# Autodesk Inventor assembly: BRUSH CAGE
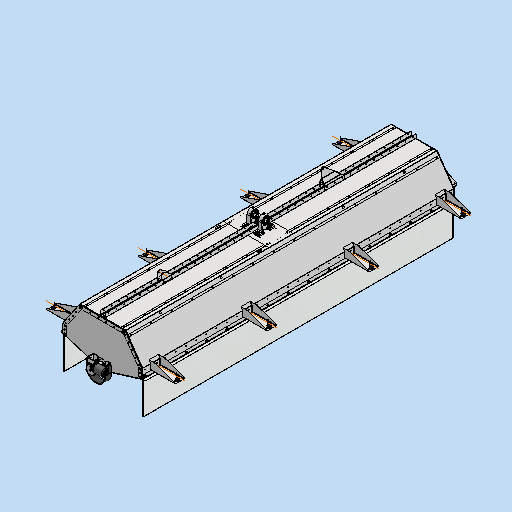
[picture p0: Inventor's stored thumbnail of the model, 512x512]
Saved by Autodesk Inventor 2025.3 (Build 293356030, 356C)
## iProperties
Created: 2025-10-16
Part Number: BRUSH CAGE
Document SubType Name: Assembly
Designer: josh
Mass: 36893.9 g
Surface Area: 125831 cm^2
Volume: 14195.9 cm^3
Density: 2.59891 g/cm^3
Description: BRUSH CAGE COMPLETE, 24" DIAMETER CLEANING BRUSH
Author: josh
## iProperties of the stored document MemberDocs/x12ie5t5mHcoruiwyIxmpz3yaDh
Created: 2025-10-16
Document SubType Name: Assembly
Designer: josh
Mass: 36893.9 g
Surface Area: 125831 cm^2
Volume: 14195.9 cm^3
Density: 2.59891 g/cm^3
Author: josh
## iProperties of the stored document MemberDocs/x01a42iyfB0kmvj1hN3chjb54Ee
Created: 2025-10-16
Document SubType Name: Assembly
Designer: josh
Mass: 36893.9 g
Surface Area: 125831 cm^2
Volume: 14195.9 cm^3
Density: 2.59891 g/cm^3
Author: josh
## iProperties of the stored document MemberDocs/xYuatkekjKkzsr2lw34jfvc5pCb
Created: 2025-10-16
Document SubType Name: Assembly
Designer: josh
Mass: 36893.9 g
Surface Area: 125831 cm^2
Volume: 14195.9 cm^3
Density: 2.59891 g/cm^3
Author: josh
## Documents named in this file (45)
- R:\A1- Neuweg Design Data\OM Robotics\CLEANING BRUSH CAGE & ROLLER\BRUSH CAGE RevC.iam
- R:\A1- Neuweg Design Data\OM Robotics\CLEANING BRUSH CAGE & ROLLER\OM_CAGE-011.ipt
- R:\A1- Neuweg Design Data\OM Robotics\CLEANING BRUSH CAGE & ROLLER\OM_CAGE-012.ipt
- R:\A1- Neuweg Design Data\OM Robotics\CLEANING BRUSH CAGE & ROLLER\OM_CAGE-013.ipt
- R:\A1- Neuweg Design Data\OM Robotics\CLEANING BRUSH CAGE & ROLLER\OM_CAGE-014.ipt
- R:\A1- Neuweg Design Data\OM Robotics\CLEANING BRUSH CAGE & ROLLER\OM_CAGE-015.ipt
- R:\A1- Neuweg Design Data\OM Robotics\CLEANING BRUSH CAGE & ROLLER\OM_CAGE-016.ipt
- R:\A1- Neuweg Design Data\OM Robotics\CLEANING BRUSH CAGE & ROLLER\OM_CAGE-018.ipt
- R:\A1- Neuweg Design Data\OM Robotics\CLEANING BRUSH CAGE & ROLLER\OM_CAGE-019.ipt
- R:\A1- Neuweg Design Data\OM Robotics\CLEANING BRUSH CAGE & ROLLER\OM_CAGE-020.ipt
- R:\A1- Neuweg Design Data\OM Robotics\CLEANING BRUSH CAGE & ROLLER\Shaft Coupler.ipt
- R:\A1- Neuweg Design Data\OM Robotics\CLEANING BRUSH CAGE & ROLLER\SENSOR BRACKET RevC.iam
- R:\A1- Neuweg Design Data\OM Robotics\CLEANING BRUSH CAGE & ROLLER\OM_CAGE-021.ipt
- R:\A1- Neuweg Design Data\OM Robotics\CLEANING BRUSH CAGE & ROLLER\OM_CAGE-022.ipt
- R:\A1- Neuweg Design Data\OM Robotics\CLEANING BRUSH CAGE & ROLLER\OM_CAGE-023.ipt
- R:\A1- Neuweg Design Data\OM Robotics\CLEANING BRUSH CAGE & ROLLER\OM_CAGE-024.ipt
- R:\A1- Neuweg Design Data\OM Robotics\CLEANING BRUSH CAGE & ROLLER\4453N16.ipt
- R:\A1- Neuweg Design Data\OM Robotics\CLEANING BRUSH CAGE & ROLLER\UCFL205-16_Simplify.ipt
- R:\A1- Neuweg Design Data\OM Robotics\CLEANING BRUSH CAGE & ROLLER\BRUSH TUBE_RevA.iam
- R:\A1- Neuweg Design Data\OM Robotics\CLEANING BRUSH CAGE & ROLLER\218-2002_Simplify.ipt
- R:\A1- Neuweg Design Data\OM Robotics\CLEANING BRUSH CAGE & ROLLER\94842A101.ipt
- R:\A1- Neuweg Design Data\OM Robotics\CLEANING BRUSH CAGE & ROLLER\95031A124.ipt
- R:\A1- Neuweg Design Data\OM Robotics\CLEANING BRUSH CAGE & ROLLER\Fan Bracket.ipt
- R:\A1- Neuweg Design Data\OM Robotics\CLEANING BRUSH CAGE & ROLLER\98778A541.ipt
- C:\WORK\INVENTOR PROJECTS\misc custom projects\O&M ROBOTICS\OM_CAGE-011.ipt
- C:\WORK\INVENTOR PROJECTS\misc custom projects\O&M ROBOTICS\OM_CAGE-012.ipt
- C:\WORK\INVENTOR PROJECTS\misc custom projects\O&M ROBOTICS\OM_CAGE-013.ipt
- C:\WORK\INVENTOR PROJECTS\misc custom projects\O&M ROBOTICS\OM_CAGE-014.ipt
- C:\WORK\INVENTOR PROJECTS\misc custom projects\O&M ROBOTICS\OM_CAGE-015.ipt
- C:\WORK\INVENTOR PROJECTS\misc custom projects\O&M ROBOTICS\OM_CAGE-016.ipt
- C:\WORK\INVENTOR PROJECTS\misc custom projects\O&M ROBOTICS\OM_CAGE-018.ipt
- C:\WORK\INVENTOR PROJECTS\misc custom projects\O&M ROBOTICS\OM_CAGE-019.ipt
- C:\WORK\INVENTOR PROJECTS\misc custom projects\O&M ROBOTICS\OM_CAGE-020.ipt
- C:\WORK\INVENTOR PROJECTS\misc custom projects\O&M ROBOTICS\ucfl205-16\ucfl205-16\ucfl205-16.iam
- C:\WORK\INVENTOR PROJECTS\misc custom projects\O&M ROBOTICS\BRUSH TUBE_RevA.iam
- C:\WORK\INVENTOR PROJECTS\misc custom projects\O&M ROBOTICS\Shaft Coupler.ipt
- C:\WORK\INVENTOR PROJECTS\misc custom projects\O&M ROBOTICS\218-2002\218-2002\218-2002.iam
- C:\WORK\INVENTOR PROJECTS\misc custom projects\O&M ROBOTICS\SENSOR BRACKET RevC.iam
- C:\WORK\INVENTOR PROJECTS\misc custom projects\O&M ROBOTICS\ucpa205-16\ucpa205-16\ucpa205-16.iam
- C:\WORK\INVENTOR PROJECTS\misc custom projects\O&M ROBOTICS\OM_CAGE-021.ipt
- C:\WORK\INVENTOR PROJECTS\misc custom projects\O&M ROBOTICS\Fan+Bracket.iam
- C:\WORK\INVENTOR PROJECTS\misc custom projects\O&M ROBOTICS\4453N16_Extra-Clearance Mounted Ball Bearing.ipt
- C:\WORK\INVENTOR PROJECTS\misc custom projects\O&M ROBOTICS\OM_CAGE-022.ipt
- C:\WORK\INVENTOR PROJECTS\misc custom projects\O&M ROBOTICS\OM_CAGE-023.ipt
- C:\WORK\INVENTOR PROJECTS\misc custom projects\O&M ROBOTICS\OM_CAGE-024.ipt
## Components (228 placed, 23 different names)
1. OM_CAGE-011:1 — Mate:4, Mate:5, Mate:6, Mate:8, Mate:10, Mate:11, Mate:18, Mate:17, Insert:16, Insert:17, Mate:20, Mate:22, Mate:23, Mate:24, Mate:25, Mate:26, Mate:27, Mate:28, Mate:29, Mate:30, Mate:31, Mate:32, Mate:33, Mate:34, Mate:35, Insert:95, Insert:96, Insert:97, Insert:98, Insert:99, Insert:100, Insert:101, Insert:102, Insert:103, Insert:104, Insert:105, Insert:106, Insert:107, Insert:108, Insert:109, Insert:110, Insert:111, Insert:112, Insert:113, Insert:114, Insert:115, Insert:116, Insert:117, Insert:118, Insert:119, Insert:120, Insert:121, Insert:122, Insert:123, Insert:124, Insert:125, Insert:126, Insert:127, Insert:128, Insert:129, Insert:130, Insert:131, Insert:132, Insert:133, Insert:134, Insert:135, Insert:136, Insert:137, Insert:138, Insert:139, Insert:140, Insert:141, Insert:142, Insert:143, Insert:144, Insert:145, Insert:146, Insert:147, Insert:148, Insert:149, Insert:150, Insert:151, Insert:152, Insert:153, Insert:154, Insert:155, Insert:156, Insert:157, Insert:158, Insert:159, Insert:160, Insert:161, Insert:162, Insert:163, Insert:164, Insert:165, Insert:166, Insert:167, Insert:168, Insert:169, Insert:170, Insert:171, Insert:172, Insert:173, Insert:174, Insert:175, Insert:176, Insert:177, Insert:178, Insert:179, Insert:180, Insert:181, Insert:182, Insert:183, Insert:184, Insert:185, Insert:186, Insert:187, Insert:188, Insert:189, Insert:190
2. OM_CAGE-012:1 — Insert:25, Insert:26, Insert:31, Insert:32, Insert:33, Insert:34, Insert:35, Insert:36, Insert:37, Insert:38, Insert:39, Insert:40, Insert:41, Insert:42, Insert:43, Insert:44, Insert:45, Insert:46, Insert:47, Insert:48, Insert:49, Insert:50, Insert:51, Insert:52
3. OM_CAGE-013:1 — Mate:15, Insert:12, Insert:13, Mate:16, Mate:19, Insert:20, Insert:21, Insert:23, Insert:24, Insert:75, Insert:76, Insert:77, Insert:78, Insert:79, Insert:80, Insert:81, Insert:82, Insert:83, Insert:84, Insert:85, Insert:86, Insert:87, Insert:88, Insert:89, Insert:90, Insert:91, Insert:92, Insert:93, Insert:94
4. OM_CAGE-014:1
5. OM_CAGE-015:1
6. OM_CAGE-016:1 — Insert:191, Insert:192, Insert:193, Insert:194, Insert:195, Insert:196, Insert:197, Insert:198, Insert:199, Insert:200, Insert:201, Insert:202, Insert:203, Insert:204, Insert:205, Insert:206
7. OM_CAGE-018:1 — Insert:11
8. OM_CAGE-019:1 — Mate:36, Insert:27, Insert:28, Insert:53, Insert:54, Insert:55, Insert:56, Insert:57, Insert:58, Insert:59, Insert:60, Insert:61, Insert:62, Insert:63, Insert:64, Insert:65, Insert:66, Insert:67, Insert:68, Insert:69, Insert:70, Insert:71, Insert:72, Insert:73, Insert:74, Flush:2, Mate:39, Mate:40, Mate:41, Mate:42, Mate:43
9. OM_CAGE-020:1
10. OM_CAGE-018:2
11. OM_CAGE-020:2
12. OM_CAGE-015:2
13. OM_CAGE-016:2 — Insert:207, Insert:208, Insert:209, Insert:210, Insert:211, Insert:212, Insert:213, Insert:214, Insert:215, Insert:216, Insert:217, Insert:218, Insert:219, Insert:220, Insert:221, Insert:222
14. UCFL205-16_Simplify:1 — Insert:25, Insert:26, Insert:29
15. UCFL205-16_Simplify:2 — Mate:36, Insert:27, Insert:28, Mate:37
16. Shaft Coupler:1 — Mate:3, Mate:38, Insert:30
17. 218-2002_Simplify:1 — Mate:3, Insert:11
18. SENSOR BRACKET RevC:1 [sub-assembly] — Mate:4, Mate:5
19. SENSOR BRACKET RevC:2 [sub-assembly] — Mate:6, Mate:26, Mate:27
20. SENSOR BRACKET RevC:3 [sub-assembly] — Mate:10, Mate:11, Mate:24, Mate:25
21. SENSOR BRACKET RevC:4 [sub-assembly] — Mate:8, Mate:22, Mate:23
22. SENSOR BRACKET RevC:5 [sub-assembly] — Mate:31, Mate:32
23. SENSOR BRACKET RevC:6 [sub-assembly] — Mate:30, Mate:33
24. SENSOR BRACKET RevC:7 [sub-assembly] — Mate:28, Mate:35
25. SENSOR BRACKET RevC:8 [sub-assembly] — Mate:29, Mate:34
26. OM_CAGE-021:1 — Mate:14, Flush:1, Insert:12, Insert:13
27. OM_CAGE-021:2 — Mate:14, Mate:15, Flush:1
28. Fan Bracket:1 — Flush:2, Mate:40, Mate:43
29. Fan Bracket:2 — Mate:39, Mate:41, Mate:42
30. 4453N16:1 — Mate:16, Mate:18, Mate:17, Mate:19, Mate:21
31. OM_CAGE-022:1
32. OM_CAGE-022:2 — Insert:16, Insert:17
33. 4453N16:2 — Mate:20, Mate:21
34. OM_CAGE-023:1 — Insert:20, Insert:21, Insert:22
35. OM_CAGE-024:1 — Insert:22, Insert:23, Insert:24
36. BRUSH TUBE_RevA:1 [sub-assembly] — Insert:29, Mate:37, Mate:38, Insert:30
37. 98778A541:1 — Insert:31
38. 98778A541:2 — Insert:32
39. 98778A541:3 — Insert:33
40. 98778A541:4 — Insert:34
41. 98778A541:5 — Insert:35
42. 98778A541:6 — Insert:36
43. 98778A541:7 — Insert:37
44. 98778A541:8 — Insert:38
45. 98778A541:9 — Insert:39
46. 98778A541:10 — Insert:40
47. 98778A541:11 — Insert:41
48. 98778A541:12 — Insert:42
49. 98778A541:13 — Insert:43
50. 98778A541:14 — Insert:44
51. 98778A541:15 — Insert:45
52. 98778A541:16 — Insert:46
53. 98778A541:17 — Insert:47
54. 98778A541:18 — Insert:48
55. 98778A541:19 — Insert:49
56. 98778A541:20 — Insert:50
57. 98778A541:21 — Insert:51
58. 98778A541:22 — Insert:52
59. 98778A541:23 — Insert:53
60. 98778A541:24 — Insert:54
61. 98778A541:25 — Insert:55
62. 98778A541:26 — Insert:56
63. 98778A541:27 — Insert:57
64. 98778A541:28 — Insert:58
65. 98778A541:29 — Insert:59
66. 98778A541:30 — Insert:60
67. 98778A541:31 — Insert:61
68. 98778A541:32 — Insert:62
69. 98778A541:33 — Insert:63
70. 98778A541:34 — Insert:64
71. 98778A541:35 — Insert:65
72. 98778A541:36 — Insert:66
73. 98778A541:37 — Insert:67
74. 98778A541:38 — Insert:68
75. 98778A541:39 — Insert:69
76. 98778A541:40 — Insert:70
77. 98778A541:41 — Insert:71
78. 98778A541:42 — Insert:72
79. 98778A541:43 — Insert:73
80. 98778A541:44 — Insert:74
81. 98778A541:45 — Insert:75
82. 98778A541:46 — Insert:76
83. 98778A541:47 — Insert:77
84. 98778A541:48 — Insert:78
85. 98778A541:49 — Insert:79
86. 98778A541:50 — Insert:80
87. 98778A541:51 — Insert:81
88. 98778A541:52 — Insert:82
89. 98778A541:53 — Insert:83
90. 98778A541:54 — Insert:84
91. 98778A541:55 — Insert:85
92. 98778A541:56 — Insert:86
93. 98778A541:57 — Insert:87
94. 98778A541:58 — Insert:88
95. 98778A541:59 — Insert:89
96. 98778A541:60 — Insert:90
97. 98778A541:61 — Insert:91
98. 98778A541:62 — Insert:92
99. 98778A541:63 — Insert:93
100. 98778A541:64 — Insert:94
101. 98778A541:65 — Insert:95
102. 98778A541:66 — Insert:96
103. 98778A541:67 — Insert:97
104. 98778A541:68 — Insert:98
105. 98778A541:69 — Insert:99
106. 98778A541:70 — Insert:100
107. 98778A541:71 — Insert:101
108. 98778A541:72 — Insert:102
109. 98778A541:73 — Insert:103
110. 98778A541:74 — Insert:104
111. 98778A541:75 — Insert:105
112. 98778A541:76 — Insert:106
113. 98778A541:77 — Insert:107
114. 98778A541:78 — Insert:108
115. 98778A541:79 — Insert:109
116. 98778A541:80 — Insert:110
117. 98778A541:81 — Insert:111
118. 98778A541:82 — Insert:112
119. 98778A541:83 — Insert:113
120. 98778A541:84 — Insert:114
121. 98778A541:85 — Insert:115
122. 98778A541:86 — Insert:116
123. 98778A541:87 — Insert:117
124. 98778A541:88 — Insert:118
125. 98778A541:89 — Insert:119
126. 98778A541:90 — Insert:120
127. 98778A541:91 — Insert:121
128. 98778A541:92 — Insert:122
129. 98778A541:93 — Insert:123
130. 98778A541:94 — Insert:124
131. 98778A541:95 — Insert:125
132. 98778A541:96 — Insert:126
133. 98778A541:97 — Insert:127
134. 98778A541:98 — Insert:128
135. 98778A541:99 — Insert:129
136. 98778A541:100 — Insert:130
137. 98778A541:101 — Insert:131
138. 98778A541:102 — Insert:132
139. 98778A541:103 — Insert:133
140. 98778A541:104 — Insert:134
141. 98778A541:105 — Insert:135
142. 98778A541:106 — Insert:136
143. 98778A541:107 — Insert:137
144. 98778A541:108 — Insert:138
145. 98778A541:109 — Insert:139
146. 98778A541:110 — Insert:140
147. 98778A541:111 — Insert:141
148. 98778A541:112 — Insert:142
149. 98778A541:113 — Insert:143
150. 98778A541:114 — Insert:144
151. 98778A541:115 — Insert:145
152. 98778A541:116 — Insert:146
153. 98778A541:117 — Insert:147
154. 98778A541:118 — Insert:148
155. 98778A541:119 — Insert:149
156. 98778A541:120 — Insert:150
157. 98778A541:121 — Insert:151
158. 98778A541:122 — Insert:152
159. 98778A541:123 — Insert:153
160. 98778A541:124 — Insert:154
161. 98778A541:125 — Insert:155
162. 98778A541:126 — Insert:156
163. 98778A541:127 — Insert:157
164. 98778A541:128 — Insert:158
165. 94842A101:1 — Insert:159
166. 94842A101:2 — Insert:160
167. 94842A101:3 — Insert:161
168. 94842A101:4 — Insert:162
169. 94842A101:5 — Insert:163
170. 94842A101:6 — Insert:164
171. 94842A101:7 — Insert:165
172. 94842A101:8 — Insert:166
173. 94842A101:9 — Insert:167
174. 94842A101:10 — Insert:168
175. 94842A101:11 — Insert:169
176. 94842A101:12 — Insert:170
177. 94842A101:13 — Insert:171
178. 94842A101:14 — Insert:172
179. 94842A101:15 — Insert:173
180. 94842A101:16 — Insert:174
181. 94842A101:17 — Insert:175
182. 94842A101:18 — Insert:176
183. 94842A101:19 — Insert:177
184. 94842A101:20 — Insert:178
185. 94842A101:21 — Insert:179
186. 94842A101:22 — Insert:180
187. 94842A101:23 — Insert:181
188. 94842A101:24 — Insert:182
189. 94842A101:25 — Insert:183
190. 94842A101:26 — Insert:184
191. 94842A101:27 — Insert:185
192. 94842A101:28 — Insert:186
193. 94842A101:29 — Insert:187
194. 94842A101:30 — Insert:188
195. 94842A101:31 — Insert:189
196. 94842A101:32 — Insert:190
197. 95031A124:1 — Insert:191
198. 95031A124:2 — Insert:192
199. 95031A124:3 — Insert:193
200. 95031A124:4 — Insert:194
201. 95031A124:5 — Insert:195
202. 95031A124:6 — Insert:196
203. 95031A124:7 — Insert:197
204. 95031A124:8 — Insert:198
205. 95031A124:9 — Insert:199
206. 95031A124:10 — Insert:200
207. 95031A124:11 — Insert:201
208. 95031A124:12 — Insert:202
209. 95031A124:13 — Insert:203
210. 95031A124:14 — Insert:204
211. 95031A124:15 — Insert:205
212. 95031A124:16 — Insert:206
213. 95031A124:17 — Insert:207
214. 95031A124:18 — Insert:208
215. 95031A124:19 — Insert:209
216. 95031A124:20 — Insert:210
217. 95031A124:21 — Insert:211
218. 95031A124:22 — Insert:212
219. 95031A124:23 — Insert:213
220. 95031A124:24 — Insert:214
221. 95031A124:25 — Insert:215
222. 95031A124:26 — Insert:216
223. 95031A124:27 — Insert:217
224. 95031A124:28 — Insert:218
225. 95031A124:29 — Insert:219
226. 95031A124:30 — Insert:220
227. 95031A124:31 — Insert:221
228. 95031A124:32 — Insert:222
## Relationships (247: Insert 208, Mate 37, Flush 2)
- Mate:3: Shaft Coupler:1 ↔ 218-2002_Simplify:1
- Mate:4: OM_CAGE-011:1 ↔ SENSOR BRACKET RevC:1
- Mate:5: OM_CAGE-011:1 ↔ SENSOR BRACKET RevC:1
- Mate:6: OM_CAGE-011:1 ↔ SENSOR BRACKET RevC:2
- Mate:8: OM_CAGE-011:1 ↔ SENSOR BRACKET RevC:4
- Mate:10: OM_CAGE-011:1 ↔ SENSOR BRACKET RevC:3
- Mate:11: OM_CAGE-011:1 ↔ SENSOR BRACKET RevC:3
- Insert:11: OM_CAGE-018:1 ↔ 218-2002_Simplify:1
- Mate:14: OM_CAGE-021:1 ↔ OM_CAGE-021:2
- Mate:15: OM_CAGE-013:1 ↔ OM_CAGE-021:2
- Flush:1: OM_CAGE-021:1 ↔ OM_CAGE-021:2
- Insert:12: OM_CAGE-013:1 ↔ OM_CAGE-021:1
- Insert:13: OM_CAGE-013:1 ↔ OM_CAGE-021:1
- Mate:16: OM_CAGE-013:1 ↔ 4453N16:1
- Mate:18: OM_CAGE-011:1 ↔ 4453N16:1
- Mate:17: OM_CAGE-011:1 ↔ 4453N16:1
- Mate:19 (0.3556 mm): OM_CAGE-013:1 ↔ 4453N16:1
- Insert:16: OM_CAGE-011:1 ↔ OM_CAGE-022:2
- Insert:17: OM_CAGE-011:1 ↔ OM_CAGE-022:2
- Mate:20: OM_CAGE-011:1 ↔ 4453N16:2
- Mate:21: 4453N16:1 ↔ 4453N16:2
- Mate:22: OM_CAGE-011:1 ↔ SENSOR BRACKET RevC:4
- Mate:23: OM_CAGE-011:1 ↔ SENSOR BRACKET RevC:4
- Mate:24: OM_CAGE-011:1 ↔ SENSOR BRACKET RevC:3
- Mate:25: OM_CAGE-011:1 ↔ SENSOR BRACKET RevC:3
- Mate:26: OM_CAGE-011:1 ↔ SENSOR BRACKET RevC:2
- Mate:27: OM_CAGE-011:1 ↔ SENSOR BRACKET RevC:2
- Mate:28: OM_CAGE-011:1 ↔ SENSOR BRACKET RevC:7
- Mate:29: OM_CAGE-011:1 ↔ SENSOR BRACKET RevC:8
- Mate:30: OM_CAGE-011:1 ↔ SENSOR BRACKET RevC:6
- Mate:31: OM_CAGE-011:1 ↔ SENSOR BRACKET RevC:5
- Mate:32: OM_CAGE-011:1 ↔ SENSOR BRACKET RevC:5
- Mate:33: OM_CAGE-011:1 ↔ SENSOR BRACKET RevC:6
- Mate:34: OM_CAGE-011:1 ↔ SENSOR BRACKET RevC:8
- Mate:35: OM_CAGE-011:1 ↔ SENSOR BRACKET RevC:7
- Insert:20: OM_CAGE-013:1 ↔ OM_CAGE-023:1
- Insert:21: OM_CAGE-013:1 ↔ OM_CAGE-023:1
- Insert:22: OM_CAGE-023:1 ↔ OM_CAGE-024:1
- Insert:23: OM_CAGE-013:1 ↔ OM_CAGE-024:1
- Insert:24: OM_CAGE-013:1 ↔ OM_CAGE-024:1
- Insert:25: OM_CAGE-012:1 ↔ UCFL205-16_Simplify:1
- Mate:36: OM_CAGE-019:1 ↔ UCFL205-16_Simplify:2
- Insert:26: OM_CAGE-012:1 ↔ UCFL205-16_Simplify:1
- Insert:27: OM_CAGE-019:1 ↔ UCFL205-16_Simplify:2
- Insert:28: OM_CAGE-019:1 ↔ UCFL205-16_Simplify:2
- Insert:29 (1.5875 mm): UCFL205-16_Simplify:1 ↔ BRUSH TUBE_RevA:1
- Mate:37: UCFL205-16_Simplify:2 ↔ BRUSH TUBE_RevA:1
- Mate:38: Shaft Coupler:1 ↔ BRUSH TUBE_RevA:1
- Insert:30: Shaft Coupler:1 ↔ BRUSH TUBE_RevA:1
- Insert:31: OM_CAGE-012:1 ↔ 98778A541:1
- Insert:32: OM_CAGE-012:1 ↔ 98778A541:2
- Insert:33: OM_CAGE-012:1 ↔ 98778A541:3
- Insert:34: OM_CAGE-012:1 ↔ 98778A541:4
- Insert:35: OM_CAGE-012:1 ↔ 98778A541:5
- Insert:36: OM_CAGE-012:1 ↔ 98778A541:6
- Insert:37: OM_CAGE-012:1 ↔ 98778A541:7
- Insert:38: OM_CAGE-012:1 ↔ 98778A541:8
- Insert:39: OM_CAGE-012:1 ↔ 98778A541:9
- Insert:40: OM_CAGE-012:1 ↔ 98778A541:10
- Insert:41: OM_CAGE-012:1 ↔ 98778A541:11
- Insert:42: OM_CAGE-012:1 ↔ 98778A541:12
- Insert:43: OM_CAGE-012:1 ↔ 98778A541:13
- Insert:44: OM_CAGE-012:1 ↔ 98778A541:14
- Insert:45: OM_CAGE-012:1 ↔ 98778A541:15
- Insert:46: OM_CAGE-012:1 ↔ 98778A541:16
- Insert:47: OM_CAGE-012:1 ↔ 98778A541:17
- Insert:48: OM_CAGE-012:1 ↔ 98778A541:18
- Insert:49: OM_CAGE-012:1 ↔ 98778A541:19
- Insert:50: OM_CAGE-012:1 ↔ 98778A541:20
- Insert:51: OM_CAGE-012:1 ↔ 98778A541:21
- Insert:52: OM_CAGE-012:1 ↔ 98778A541:22
- Insert:53: OM_CAGE-019:1 ↔ 98778A541:23
- Insert:54: OM_CAGE-019:1 ↔ 98778A541:24
- Insert:55: OM_CAGE-019:1 ↔ 98778A541:25
- Insert:56: OM_CAGE-019:1 ↔ 98778A541:26
- Insert:57: OM_CAGE-019:1 ↔ 98778A541:27
- Insert:58: OM_CAGE-019:1 ↔ 98778A541:28
- Insert:59: OM_CAGE-019:1 ↔ 98778A541:29
- Insert:60: OM_CAGE-019:1 ↔ 98778A541:30
- Insert:61: OM_CAGE-019:1 ↔ 98778A541:31
- Insert:62: OM_CAGE-019:1 ↔ 98778A541:32
- Insert:63: OM_CAGE-019:1 ↔ 98778A541:33
- Insert:64: OM_CAGE-019:1 ↔ 98778A541:34
- Insert:65: OM_CAGE-019:1 ↔ 98778A541:35
- Insert:66: OM_CAGE-019:1 ↔ 98778A541:36
- Insert:67: OM_CAGE-019:1 ↔ 98778A541:37
- Insert:68: OM_CAGE-019:1 ↔ 98778A541:38
- Insert:69: OM_CAGE-019:1 ↔ 98778A541:39
- Insert:70: OM_CAGE-019:1 ↔ 98778A541:40
- Insert:71: OM_CAGE-019:1 ↔ 98778A541:41
- Insert:72: OM_CAGE-019:1 ↔ 98778A541:42
- Insert:73: OM_CAGE-019:1 ↔ 98778A541:43
- Insert:74: OM_CAGE-019:1 ↔ 98778A541:44
- Insert:75: OM_CAGE-013:1 ↔ 98778A541:45
- Insert:76: OM_CAGE-013:1 ↔ 98778A541:46
- Insert:77: OM_CAGE-013:1 ↔ 98778A541:47
- Insert:78: OM_CAGE-013:1 ↔ 98778A541:48
- Insert:79: OM_CAGE-013:1 ↔ 98778A541:49
- Insert:80: OM_CAGE-013:1 ↔ 98778A541:50
- Insert:81: OM_CAGE-013:1 ↔ 98778A541:51
- Insert:82: OM_CAGE-013:1 ↔ 98778A541:52
- Insert:83: OM_CAGE-013:1 ↔ 98778A541:53
- Insert:84: OM_CAGE-013:1 ↔ 98778A541:54
- Insert:85: OM_CAGE-013:1 ↔ 98778A541:55
- Insert:86: OM_CAGE-013:1 ↔ 98778A541:56
- Insert:87: OM_CAGE-013:1 ↔ 98778A541:57
- Insert:88: OM_CAGE-013:1 ↔ 98778A541:58
- Insert:89: OM_CAGE-013:1 ↔ 98778A541:59
- Insert:90: OM_CAGE-013:1 ↔ 98778A541:60
- Insert:91: OM_CAGE-013:1 ↔ 98778A541:61
- Insert:92: OM_CAGE-013:1 ↔ 98778A541:62
- Insert:93: OM_CAGE-013:1 ↔ 98778A541:63
- Insert:94: OM_CAGE-013:1 ↔ 98778A541:64
- Insert:95: OM_CAGE-011:1 ↔ 98778A541:65
- Insert:96: OM_CAGE-011:1 ↔ 98778A541:66
- Insert:97: OM_CAGE-011:1 ↔ 98778A541:67
- Insert:98: OM_CAGE-011:1 ↔ 98778A541:68
- Insert:99: OM_CAGE-011:1 ↔ 98778A541:69
- Insert:100: OM_CAGE-011:1 ↔ 98778A541:70
- Insert:101: OM_CAGE-011:1 ↔ 98778A541:71
- Insert:102: OM_CAGE-011:1 ↔ 98778A541:72
- Insert:103: OM_CAGE-011:1 ↔ 98778A541:73
- Insert:104: OM_CAGE-011:1 ↔ 98778A541:74
- Insert:105: OM_CAGE-011:1 ↔ 98778A541:75
- Insert:106: OM_CAGE-011:1 ↔ 98778A541:76
- Insert:107: OM_CAGE-011:1 ↔ 98778A541:77
- Insert:108: OM_CAGE-011:1 ↔ 98778A541:78
- Insert:109: OM_CAGE-011:1 ↔ 98778A541:79
- Insert:110: OM_CAGE-011:1 ↔ 98778A541:80
- Insert:111: OM_CAGE-011:1 ↔ 98778A541:81
- Insert:112: OM_CAGE-011:1 ↔ 98778A541:82
- Insert:113: OM_CAGE-011:1 ↔ 98778A541:83
- Insert:114: OM_CAGE-011:1 ↔ 98778A541:84
- Insert:115: OM_CAGE-011:1 ↔ 98778A541:85
- Insert:116: OM_CAGE-011:1 ↔ 98778A541:86
- Insert:117: OM_CAGE-011:1 ↔ 98778A541:87
- Insert:118: OM_CAGE-011:1 ↔ 98778A541:88
- Insert:119: OM_CAGE-011:1 ↔ 98778A541:89
- Insert:120: OM_CAGE-011:1 ↔ 98778A541:90
- Insert:121: OM_CAGE-011:1 ↔ 98778A541:91
- Insert:122: OM_CAGE-011:1 ↔ 98778A541:92
- Insert:123: OM_CAGE-011:1 ↔ 98778A541:93
- Insert:124: OM_CAGE-011:1 ↔ 98778A541:94
- Insert:125: OM_CAGE-011:1 ↔ 98778A541:95
- Insert:126: OM_CAGE-011:1 ↔ 98778A541:96
- Insert:127: OM_CAGE-011:1 ↔ 98778A541:97
- Insert:128: OM_CAGE-011:1 ↔ 98778A541:98
- Insert:129: OM_CAGE-011:1 ↔ 98778A541:99
- Insert:130: OM_CAGE-011:1 ↔ 98778A541:100
- Insert:131: OM_CAGE-011:1 ↔ 98778A541:101
- Insert:132: OM_CAGE-011:1 ↔ 98778A541:102
- Insert:133: OM_CAGE-011:1 ↔ 98778A541:103
- Insert:134: OM_CAGE-011:1 ↔ 98778A541:104
- Insert:135: OM_CAGE-011:1 ↔ 98778A541:105
- Insert:136: OM_CAGE-011:1 ↔ 98778A541:106
- Insert:137: OM_CAGE-011:1 ↔ 98778A541:107
- Insert:138: OM_CAGE-011:1 ↔ 98778A541:108
- Insert:139: OM_CAGE-011:1 ↔ 98778A541:109
- Insert:140: OM_CAGE-011:1 ↔ 98778A541:110
- Insert:141: OM_CAGE-011:1 ↔ 98778A541:111
- Insert:142: OM_CAGE-011:1 ↔ 98778A541:112
- Insert:143: OM_CAGE-011:1 ↔ 98778A541:113
- Insert:144: OM_CAGE-011:1 ↔ 98778A541:114
- Insert:145: OM_CAGE-011:1 ↔ 98778A541:115
- Insert:146: OM_CAGE-011:1 ↔ 98778A541:116
- Insert:147: OM_CAGE-011:1 ↔ 98778A541:117
- Insert:148: OM_CAGE-011:1 ↔ 98778A541:118
- Insert:149: OM_CAGE-011:1 ↔ 98778A541:119
- Insert:150: OM_CAGE-011:1 ↔ 98778A541:120
- Insert:151: OM_CAGE-011:1 ↔ 98778A541:121
- Insert:152: OM_CAGE-011:1 ↔ 98778A541:122
- Insert:153: OM_CAGE-011:1 ↔ 98778A541:123
- Insert:154: OM_CAGE-011:1 ↔ 98778A541:124
- Insert:155: OM_CAGE-011:1 ↔ 98778A541:125
- Insert:156: OM_CAGE-011:1 ↔ 98778A541:126
- Insert:157: OM_CAGE-011:1 ↔ 98778A541:127
- Insert:158: OM_CAGE-011:1 ↔ 98778A541:128
- Insert:159: OM_CAGE-011:1 ↔ 94842A101:1
- Insert:160: OM_CAGE-011:1 ↔ 94842A101:2
- Insert:161: OM_CAGE-011:1 ↔ 94842A101:3
- Insert:162: OM_CAGE-011:1 ↔ 94842A101:4
- Insert:163: OM_CAGE-011:1 ↔ 94842A101:5
- Insert:164: OM_CAGE-011:1 ↔ 94842A101:6
- Insert:165: OM_CAGE-011:1 ↔ 94842A101:7
- Insert:166: OM_CAGE-011:1 ↔ 94842A101:8
- Insert:167: OM_CAGE-011:1 ↔ 94842A101:9
- Insert:168: OM_CAGE-011:1 ↔ 94842A101:10
- Insert:169: OM_CAGE-011:1 ↔ 94842A101:11
- Insert:170: OM_CAGE-011:1 ↔ 94842A101:12
- Insert:171: OM_CAGE-011:1 ↔ 94842A101:13
- Insert:172: OM_CAGE-011:1 ↔ 94842A101:14
- Insert:173: OM_CAGE-011:1 ↔ 94842A101:15
- Insert:174: OM_CAGE-011:1 ↔ 94842A101:16
- Insert:175: OM_CAGE-011:1 ↔ 94842A101:17
- Insert:176: OM_CAGE-011:1 ↔ 94842A101:18
- Insert:177: OM_CAGE-011:1 ↔ 94842A101:19
- Insert:178: OM_CAGE-011:1 ↔ 94842A101:20
- Insert:179: OM_CAGE-011:1 ↔ 94842A101:21
- Insert:180: OM_CAGE-011:1 ↔ 94842A101:22
- Insert:181: OM_CAGE-011:1 ↔ 94842A101:23
- Insert:182: OM_CAGE-011:1 ↔ 94842A101:24
- Insert:183: OM_CAGE-011:1 ↔ 94842A101:25
- Insert:184: OM_CAGE-011:1 ↔ 94842A101:26
- Insert:185: OM_CAGE-011:1 ↔ 94842A101:27
- Insert:186: OM_CAGE-011:1 ↔ 94842A101:28
- Insert:187: OM_CAGE-011:1 ↔ 94842A101:29
- Insert:188: OM_CAGE-011:1 ↔ 94842A101:30
- Insert:189: OM_CAGE-011:1 ↔ 94842A101:31
- Insert:190: OM_CAGE-011:1 ↔ 94842A101:32
- Insert:191: OM_CAGE-016:1 ↔ 95031A124:1
- Insert:192: OM_CAGE-016:1 ↔ 95031A124:2
- Insert:193: OM_CAGE-016:1 ↔ 95031A124:3
- Insert:194: OM_CAGE-016:1 ↔ 95031A124:4
- Insert:195: OM_CAGE-016:1 ↔ 95031A124:5
- Insert:196: OM_CAGE-016:1 ↔ 95031A124:6
- Insert:197: OM_CAGE-016:1 ↔ 95031A124:7
- Insert:198: OM_CAGE-016:1 ↔ 95031A124:8
- Insert:199: OM_CAGE-016:1 ↔ 95031A124:9
- Insert:200: OM_CAGE-016:1 ↔ 95031A124:10
- Insert:201: OM_CAGE-016:1 ↔ 95031A124:11
- Insert:202: OM_CAGE-016:1 ↔ 95031A124:12
- Insert:203: OM_CAGE-016:1 ↔ 95031A124:13
- Insert:204: OM_CAGE-016:1 ↔ 95031A124:14
- Insert:205: OM_CAGE-016:1 ↔ 95031A124:15
- Insert:206: OM_CAGE-016:1 ↔ 95031A124:16
- Insert:207: OM_CAGE-016:2 ↔ 95031A124:17
- Insert:208: OM_CAGE-016:2 ↔ 95031A124:18
- Insert:209: OM_CAGE-016:2 ↔ 95031A124:19
- Insert:210: OM_CAGE-016:2 ↔ 95031A124:20
- Insert:211: OM_CAGE-016:2 ↔ 95031A124:21
- Insert:212: OM_CAGE-016:2 ↔ 95031A124:22
- Insert:213: OM_CAGE-016:2 ↔ 95031A124:23
- Insert:214: OM_CAGE-016:2 ↔ 95031A124:24
- Insert:215: OM_CAGE-016:2 ↔ 95031A124:25
- Insert:216: OM_CAGE-016:2 ↔ 95031A124:26
- Insert:217: OM_CAGE-016:2 ↔ 95031A124:27
- Insert:218: OM_CAGE-016:2 ↔ 95031A124:28
- Insert:219: OM_CAGE-016:2 ↔ 95031A124:29
- Insert:220: OM_CAGE-016:2 ↔ 95031A124:30
- Insert:221: OM_CAGE-016:2 ↔ 95031A124:31
- Insert:222: OM_CAGE-016:2 ↔ 95031A124:32
- Flush:2: OM_CAGE-019:1 ↔ Fan Bracket:1
- Mate:39: OM_CAGE-019:1 ↔ Fan Bracket:2
- Mate:40: OM_CAGE-019:1 ↔ Fan Bracket:1
- Mate:41: OM_CAGE-019:1 ↔ Fan Bracket:2
- Mate:42: OM_CAGE-019:1 ↔ Fan Bracket:2
- Mate:43: OM_CAGE-019:1 ↔ Fan Bracket:1
